# Autodesk Inventor assembly: KB33-046-002 - Рама
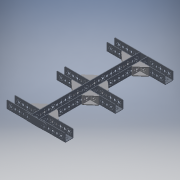
[picture p0: Inventor's stored thumbnail of the model, 180x180]
Saved by Autodesk Inventor 2019 (Build 230136000, 136)
## iProperties
Created: 2021-06-09
Part Number: KB33-046-002 - Рама
Material: Типовые
Document SubType Name: Assembly
Designer: Петров Иван
Author: Петров Иван
## Documents named in this file (3)
- E:\IVAN\Ivan_desktop\Kvantorium\Projects\RoboPatrol\design\KB33-046-001 - Ходовая часть.iam
- E:\IVAN\Ivan_desktop\Kvantorium\Projects\RoboPatrol\design\KB33-046-002 - Рама.iam
- E:\IVAN\Ivan_desktop\Kvantorium\Projects\RoboPatrol\design\KB33-046-003 - Статичный модуль мотора в сборе.iam
## Components (2 placed, 2 different names)
1. KB33-046-002 - Рама:1 [sub-assembly] — Mate:1, Mate:2, Mate:3
2. KB33-046-003 - Статичный модуль мотора в сборе:1 [sub-assembly] — Mate:1, Mate:2, Mate:3
## Relationships (3: Mate 3)
- Mate:1: KB33-046-002 - Рама:1 ↔ KB33-046-003 - Статичный модуль мотора в сборе:1
- Mate:2: KB33-046-002 - Рама:1 ↔ KB33-046-003 - Статичный модуль мотора в сборе:1
- Mate:3 (0.5 mm): KB33-046-002 - Рама:1 ↔ KB33-046-003 - Статичный модуль мотора в сборе:1
